# Autodesk Inventor assembly: onTelMountingAssy
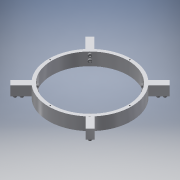
[picture p0: Inventor's stored thumbnail of the model, 180x180]
Saved by Autodesk Inventor 2016 SP1 (Build 200210100, 210)
## iProperties
Created: 2015-12-10
Part Number: onTelMountingAssy
Document SubType Name: Assembly
Designer: Dave
Author: Dave
## Documents named in this file (4)
- C:\Users\ddeboer\Desktop\leuschner-cad\onTelMountingAssy.iam
- C:\Users\ddeboer\Desktop\leuschner-cad\ontelMounting.ipt
- C:\Users\ddeboer\Desktop\leuschner-cad\mountingStub.ipt
- C:\Users\ddeboer\Desktop\leuschner-cad\qtr20_75.ipt
## Components (21 placed, 3 different names)
1. ontelMounting:1 — Flush:1
2. qtr20_75:1 — Insert:1
3. qtr20_75:2 — Insert:2
4. mountingStub:1 — Flush:1, Insert:1, Insert:2, Insert:3, Insert:4
5. qtr20_75:4 — Insert:3
6. qtr20_75:3 — Insert:4
7. qtr20_75:5
8. qtr20_75:6
9. mountingStub:2
10. qtr20_75:7
11. qtr20_75:8
12. qtr20_75:9
13. qtr20_75:10
14. mountingStub:3
15. qtr20_75:11
16. qtr20_75:12
17. qtr20_75:13
18. qtr20_75:14
19. mountingStub:4
20. qtr20_75:15
21. qtr20_75:16
## Component patterns: (4 elements, first: qtr20_75:1 + qtr20_75:2 + mountingStub:1 + qtr20_75:4 + qtr20_75:3)
## Relationships (5: Insert 4, Flush 1)
- Flush:1: ontelMounting:1 ↔ mountingStub:1
- Insert:1 (16.51 mm): qtr20_75:1 ↔ mountingStub:1
- Insert:2 (16.51 mm): qtr20_75:2 ↔ mountingStub:1
- Insert:3 (3.175 mm): mountingStub:1 ↔ qtr20_75:4
- Insert:4 (3.175 mm): mountingStub:1 ↔ qtr20_75:3
